# Autodesk Inventor assembly: Assembly12
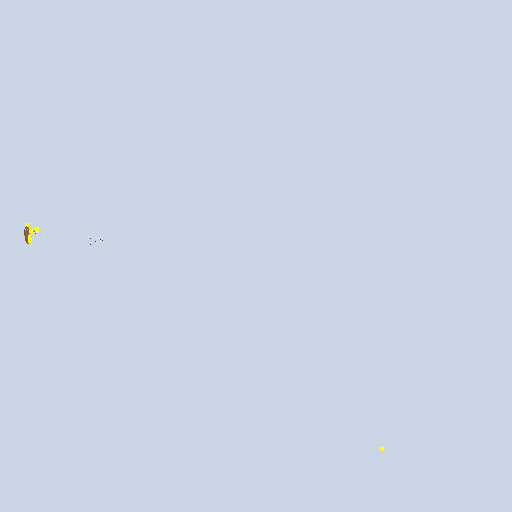
[picture p0: Inventor's stored thumbnail of the model, 512x512]
Saved by Autodesk Inventor 2024.1 (Build 281209000, 209)
## iProperties
Created: 2023-11-10
Part Number: Assembly12
Document SubType Name: Assembly
Designer: luvag
Author: luvag
## Documents named in this file (3)
- C:\Users\luvag\Desktop\Assembly12.iam
- C:\Users\luvag\Desktop\Maitri_chair.ipt
- C:\Users\luvag\Desktop\Assembly11.iam
## Components (2 placed, 2 different names)
1. Maitri_chair:1
2. Assembly11:1 [sub-assembly]
## Relationships (1: Mate 1)
- [Mate] (254 mm): Maitri_chair:1 ↔ Assembly11:1
